# Autodesk Inventor assembly: ChainInventorStudio
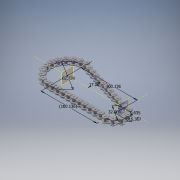
[picture p0: Inventor's stored thumbnail of the model, 180x180]
Saved by Autodesk Inventor 2016 (Build 200138000, 138)
## iProperties
Created: 2016-10-03
Part Number: ChainInventorStudio
Document SubType Name: Assembly
Designer: Kevin G
Author: Kevin G
## Documents named in this file (3)
- C:\Users\Kevin G\Documents\Inventor\KevinProject\ChainInventorStudio.iam
- C:\Users\Kevin G\Documents\Inventor\KevinProject\Master.ipt
- C:\Users\Kevin G\Documents\Inventor\KevinProject\HalfLink.ipt
## Components (38 placed, 2 different names)
1. Master:1 — Flush:1, Flush:2, Flush:3, Mate:1, Mate:2
2. HalfLink:1 — Mate:2, Mate:3, Angle:1
3. HalfLink:2
4. HalfLink:3
5. HalfLink:4
6. HalfLink:5
7. HalfLink:6
8. HalfLink:7
9. HalfLink:8
10. HalfLink:9
11. HalfLink:10
12. HalfLink:11
13. HalfLink:12
14. HalfLink:13
15. HalfLink:14
16. HalfLink:15
17. HalfLink:16
18. HalfLink:17
19. HalfLink:18
20. HalfLink:19
21. HalfLink:20
22. HalfLink:21
23. HalfLink:22
24. HalfLink:23
25. HalfLink:24
26. HalfLink:25
27. HalfLink:26
28. HalfLink:27
29. HalfLink:28
30. HalfLink:29
31. HalfLink:30
32. HalfLink:31
33. HalfLink:32
34. HalfLink:33
35. HalfLink:34
36. HalfLink:35
37. HalfLink:36
38. HalfLink:37
## Component patterns: (37 elements, first: HalfLink:1)
## Relationships (7: Flush 3, Mate 3, Angle 1)
- Flush:1: Master:1
- Flush:2: Master:1
- Flush:3: Master:1
- Mate:1 (100.136 mm): Master:1
- Mate:2: Master:1 ↔ HalfLink:1
- Mate:3: HalfLink:1
- Angle:1 (0 deg): HalfLink:1
